# Autodesk Inventor assembly: cylinder_452500010050_010754_0
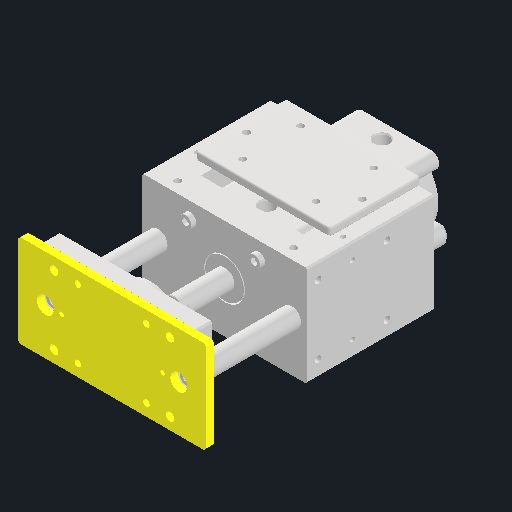
[picture p0: Inventor's stored thumbnail of the model, 512x512]
Saved by Autodesk Inventor 2025 (Build 290162000, 162)
## iProperties
Company: TraceParts S.A.
Created: 2024-05-27
Part Number: cylinder_452500010050_010754_0
Checked By: TraceParts S.A.
Catalog Web Link: www.traceparts.com
Document SubType Name: Assembly
Designer: TraceParts
Sending System: TraceParts v2
Major Version: 6.0
Minor Version: 0.0
Format Version: 0.0
Product Id: TraceParts v2
REFERENCE: 452500010050 010754
SUPPLIER: ASCO
DESIGN: 'U' guiding unit with 4 slide bearings suitable for cylinder ISO 15552-AFNOR-DIN, Ø 32 to 100 mm - 452 series - Type PLS-DM (with profiled barrel), alésage de 100 mm, course de 50 mm, Rod in Hard chrome plated steel
TraceParts.PartNumber: 10-22042010-075514
TraceParts.PartTitle: 'U' guiding unit with 4 slide bearings suitable for cylinder ISO 15552-AFNOR-DIN, Ø 32 to 100 mm - 452 series - Type PLS-DM (with profiled barrel)
TraceParts.InstanceId: 10-22042010-075514CH04KBA6VC8J3V6LU92GADS3F
TRACEPARTS: TRACEPARTS
TraceParts.PartLanguage: en
TraceParts.PartVersion: 1.3.5
Author: TraceParts
## Documents named in this file (8)
- D:\UNAL\2024-1S\APM\Digital Factory\Pneumatic Cylinders and Guides\cylinder_452500010050_010754_0.iam
- D:\UNAL\2024-1S\APM\Digital Factory\Pneumatic Cylinders and Guides\cylinder_452500010050_010754_0_01.ipt
- D:\UNAL\2024-1S\APM\Digital Factory\Pneumatic Cylinders and Guides\cylinder_452500010050_010754_0_02.ipt
- D:\UNAL\2024-1S\APM\Digital Factory\Pneumatic Cylinders and Guides\cylinder_452500010050_010754_0_03.ipt
- D:\UNAL\2024-1S\APM\Digital Factory\Pneumatic Cylinders and Guides\cylinder_452500010050_010754_0_04.ipt
- D:\UNAL\2024-1S\APM\Digital Factory\Pneumatic Cylinders and Guides\cylinder_452500010050_010754_0_05.ipt
- D:\UNAL\2024-1S\APM\Digital Factory\Packaging Machine\CylinderSupport.ipt
- D:\UNAL\2024-1S\APM\Digital Factory\Packaging Machine\TilesGrip.ipt
## Components (7 placed, 7 different names)
1. cylinder_452500010050_010754_0_Temp_1:1 — Cylindrical:1
2. cylinder_452500010050_010754_0_Temp_2:1 — Rigid:1, Cylindrical:1
3. cylinder_452500010050_010754_0_Temp_3:1 — Rigid:1, Rigid:2
4. cylinder_452500010050_010754_0_Temp_4:1 — Cylindrical:2, Flush:1
5. cylinder_452500010050_010754_0_Temp_5:1 — Rigid:2, Cylindrical:2, Flush:2
6. CylinderSupport:1 — Flush:1
7. TilesGrip:1 — Flush:2
## Relationships (6: WeldJoint 2, CylindricalJoint 2, Flush 2)
- Rigid:1 [WeldJoint]: cylinder_452500010050_010754_0_Temp_2:1 ↔ cylinder_452500010050_010754_0_Temp_3:1
- Rigid:2 [WeldJoint]: cylinder_452500010050_010754_0_Temp_3:1 ↔ cylinder_452500010050_010754_0_Temp_5:1
- Cylindrical:1: cylinder_452500010050_010754_0_Temp_1:1 ↔ cylinder_452500010050_010754_0_Temp_2:1
- Cylindrical:2: cylinder_452500010050_010754_0_Temp_4:1 ↔ cylinder_452500010050_010754_0_Temp_5:1
- Flush:1: cylinder_452500010050_010754_0_Temp_4:1 ↔ CylinderSupport:1
- Flush:2: cylinder_452500010050_010754_0_Temp_5:1 ↔ TilesGrip:1
